# Autodesk Inventor assembly: POM_T5_02_hanakawa
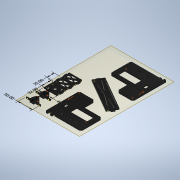
[picture p0: Inventor's stored thumbnail of the model, 180x180]
Saved by Autodesk Inventor 2022 (Build 260153000, 153)
## iProperties
Created: 2022-09-28
Part Number: POM_T5_02_hanakawa
Document SubType Name: Assembly
Designer: Masato
Author: Masato
## Documents named in this file (7)
- C:\Users\hanak\Documents\SUSTAINA-OP\Cam\POM_T5\POM_T5_02_hanakawa.iam
- C:\Users\hanak\Documents\SUSTAINA-OP\Cam\DisposableBoard.ipt
- C:\Users\hanak\Documents\SUSTAINA-OP\UpperBody\Head\Camera_side_frame.ipt
- C:\Users\hanak\Documents\SUSTAINA-OP\UpperBody\Head\Head_horn_frame.ipt
- C:\Users\hanak\Documents\SUSTAINA-OP\UpperBody\Head\Head_diagonal.ipt
- C:\Users\hanak\Documents\SUSTAINA-OP\UpperBody\Cockpit\Cockpit_battery_front_frame.ipt
- C:\Users\hanak\Documents\SUSTAINA-OP\UpperBody\Cockpit\Cockpit_side_frame.ipt
## Components (9 placed, 6 different names)
1. DisposableBoard:1 — フラッシュ:1, フラッシュ:2, フラッシュ:3, フラッシュ:4, メイト:1, メイト:2, メイト:3, メイト:4, メイト:5, メイト:6, メイト:7, メイト:9, フラッシュ:5, フラッシュ:6, メイト:10, フラッシュ:7, フラッシュ:8, メイト:11, メイト:12, メイト:13
2. Head_horn_frame:1 — メイト:4, メイト:5, 正接:1, メイト:8
3. Cockpit_side_frame:1 — メイト:9, フラッシュ:5, フラッシュ:6
4. Cockpit_side_frame:2 — メイト:10, フラッシュ:7, フラッシュ:8, 角度:1
5. Cockpit_battery_front_frame:1 — メイト:11, 角度:1, メイト:12, メイト:13
6. Camera_side_frame:1 — メイト:1, メイト:2, メイト:3
7. Camera_side_frame:2 — 正接:1
8. Head_diagonal:1 — メイト:6, メイト:7, メイト:8
9. Head_diagonal:2
## Component patterns: (2 elements, first: Camera_side_frame:1), (2 elements, first: Head_diagonal:1)
## Relationships (23: Mate 13, Flush 8, Tangent 1, Angle 1)
- フラッシュ:1 [Flush]: DisposableBoard:1
- フラッシュ:2 [Flush]: DisposableBoard:1
- フラッシュ:3 [Flush]: DisposableBoard:1
- フラッシュ:4 [Flush]: DisposableBoard:1
- メイト:1 [Mate]: DisposableBoard:1 ↔ Camera_side_frame:1
- メイト:2 [Mate] (1.5 mm): DisposableBoard:1 ↔ Camera_side_frame:1
- メイト:3 [Mate] (1.5 mm): DisposableBoard:1 ↔ Camera_side_frame:1
- メイト:4 [Mate]: DisposableBoard:1 ↔ Head_horn_frame:1
- メイト:5 [Mate] (1.5 mm): DisposableBoard:1 ↔ Head_horn_frame:1
- 正接:1 [Tangent] (3 mm): Head_horn_frame:1 ↔ Camera_side_frame:2
- メイト:6 [Mate]: DisposableBoard:1 ↔ Head_diagonal:1
- メイト:7 [Mate] (1.5 mm): DisposableBoard:1 ↔ Head_diagonal:1
- メイト:8 [Mate] (3 mm): Head_horn_frame:1 ↔ Head_diagonal:1
- メイト:9 [Mate]: DisposableBoard:1 ↔ Cockpit_side_frame:1
- フラッシュ:5 [Flush] (2.5 mm): DisposableBoard:1 ↔ Cockpit_side_frame:1
- フラッシュ:6 [Flush] (2.5 mm): DisposableBoard:1 ↔ Cockpit_side_frame:1
- メイト:10 [Mate]: DisposableBoard:1 ↔ Cockpit_side_frame:2
- フラッシュ:7 [Flush] (2.5 mm): DisposableBoard:1 ↔ Cockpit_side_frame:2
- フラッシュ:8 [Flush] (2.5 mm): DisposableBoard:1 ↔ Cockpit_side_frame:2
- メイト:11 [Mate]: DisposableBoard:1 ↔ Cockpit_battery_front_frame:1
- 角度:1 [Angle] (150 deg): Cockpit_side_frame:2 ↔ Cockpit_battery_front_frame:1
- メイト:12 [Mate] (-19 mm): DisposableBoard:1 ↔ Cockpit_battery_front_frame:1
- メイト:13 [Mate] (-173 mm): DisposableBoard:1 ↔ Cockpit_battery_front_frame:1
